# Autodesk Inventor assembly: tractionwheel_MIR
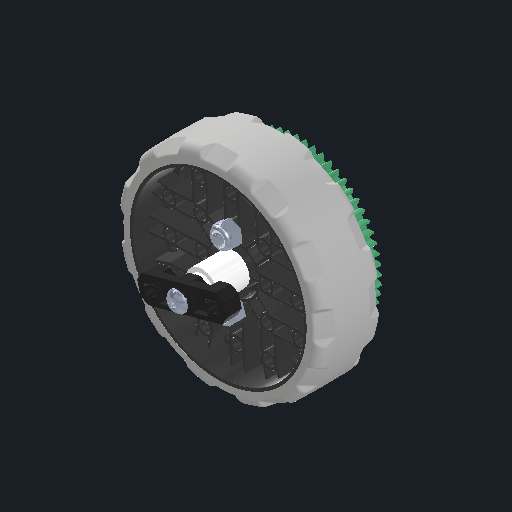
[picture p0: Inventor's stored thumbnail of the model, 512x512]
Saved by Autodesk Inventor 2024 (Build 280153000, 153)
## iProperties
Created: 2023-08-09
Part Number: tractionwheel_MIR
Document SubType Name: Assembly
Designer: macbook
Author: macbook
## Documents named in this file (16)
- \\Mac\Home\Desktop\code\1599V-VRC\Cad\Assembly\v3\tractionwheel_MIR.iam
- \\Mac\Home\Desktop\code\1599V-VRC\Cad\Motion\Shaft LS\Bearing Flat_MIR7.ipt
- \\Mac\Home\Desktop\code\1599V-VRC\Cad\Structure\Hardware\Screw Steel - Star\SScrew Star Threaded 1.250.ipt
- \\Mac\Home\Desktop\code\1599V-VRC\Cad\Structure\Hardware\Screw Steel - Star.ipt
- \\Mac\Home\Desktop\code\1599V-VRC\Cad\Structure\Hardware\Nut Nylock_MIR7.ipt
- \\Mac\Home\Desktop\code\1599V-VRC\Cad\Motion\Gears\LS 60T Gear_MIR5.ipt
- \\Mac\Home\Desktop\code\1599V-VRC\Cad\Structure\Hardware\Screw Steel - Star\SScrew Star Smooth 2.500.ipt
- \\Mac\Home\Desktop\code\1599V-VRC\Cad\Motion\Spacers\Spacer Nylon .500 OD\NSpacer White .500 OD x .500.ipt
- \\Mac\Home\Desktop\code\1599V-VRC\Cad\Motion\Spacers\Spacer Nylon .500 OD.ipt
- \\Mac\Home\Desktop\code\1599V-VRC\Cad\Motion\Spacers\Washer Steel\SWasher .375 OD x .015625.ipt
- \\Mac\Home\Desktop\code\1599V-VRC\Cad\Motion\Spacers\Washer Steel.ipt
- \\Mac\Home\Desktop\code\1599V-VRC\Cad\Motion\Spacers\Spacer Nylon .500 OD\NSpacer White .500 OD x .375.ipt
- \\Mac\Home\Desktop\code\1599V-VRC\Cad\Motion\Spacers\Washer Teflon\TWasher .375 OD x .03125.ipt
- \\Mac\Home\Desktop\code\1599V-VRC\Cad\Motion\Spacers\Washer Teflon.ipt
- \\Mac\Home\Desktop\code\1599V-VRC\Cad\Motion\Wheels\Traction Wheel\3.25 Traction AS, Circle_MIR2.iam
- \\Mac\Home\Desktop\code\1599V-VRC\Cad\Motion\Spacers\Washer Teflon\TWasher .375 OD x .06250.ipt
## Components (18 placed, 11 different names)
1. Bearing Flat_MIR7:1 — Insert:3, Insert:2, Insert:6
2. Bearing Flat_MIR7:2 — Insert:3, Insert:2, Insert:5, Insert:30
3. SScrew Star Threaded 1.250:1 — Insert:9
4. Nut Nylock_MIR7:1 — Insert:28
5. Nut Nylock_MIR7:2 — Insert:25
6. SScrew Star Threaded 1.250:2 — Insert:11
7. LS 60T Gear_MIR5:1 — Insert:29, Insert:10, Insert:12, Insert:13, Insert:27
8. SScrew Star Smooth 2.500:3 — Insert:5
9. Nut Nylock_MIR7:3 — Insert:6
10. NSpacer White .500 OD x .500:1 — Insert:22, Insert:26
11. SWasher .375 OD x .015625:1 — Insert:7
12. NSpacer White .500 OD x .375:2 — Insert:29, Insert:7, Insert:23
13. TWasher .375 OD x .03125:1 — Insert:10, Insert:9
14. TWasher .375 OD x .03125:2 — Insert:11, Insert:12
15. NSpacer White .500 OD x .375:3 — Insert:13, Insert:24
16. 3.25 Traction AS, Circle_MIR2:1 [sub-assembly] — Insert:28, Insert:25, Insert:24, Insert:23, Insert:22
17. TWasher .375 OD x .06250:3 — Insert:27
18. TWasher .375 OD x .06250:4 — Insert:30, Insert:26
## Relationships (19: Insert 19)
- Insert:3 (44.45 mm): Bearing Flat_MIR7:1 ↔ Bearing Flat_MIR7:2
- Insert:2 (44.45 mm): Bearing Flat_MIR7:1 ↔ Bearing Flat_MIR7:2
- Insert:5 (1.5875 mm): Bearing Flat_MIR7:2 ↔ SScrew Star Smooth 2.500:3
- Insert:6: Bearing Flat_MIR7:1 ↔ Nut Nylock_MIR7:3
- Insert:29: LS 60T Gear_MIR5:1 ↔ NSpacer White .500 OD x .375:2
- Insert:7: SWasher .375 OD x .015625:1 ↔ NSpacer White .500 OD x .375:2
- Insert:10: LS 60T Gear_MIR5:1 ↔ TWasher .375 OD x .03125:1
- Insert:9: SScrew Star Threaded 1.250:1 ↔ TWasher .375 OD x .03125:1
- Insert:11: SScrew Star Threaded 1.250:2 ↔ TWasher .375 OD x .03125:2
- Insert:12: LS 60T Gear_MIR5:1 ↔ TWasher .375 OD x .03125:2
- Insert:13: LS 60T Gear_MIR5:1 ↔ NSpacer White .500 OD x .375:3
- Insert:28: Nut Nylock_MIR7:1 ↔ 3.25 Traction AS, Circle_MIR2:1
- Insert:25: Nut Nylock_MIR7:2 ↔ 3.25 Traction AS, Circle_MIR2:1
- Insert:24: NSpacer White .500 OD x .375:3 ↔ 3.25 Traction AS, Circle_MIR2:1
- Insert:23: NSpacer White .500 OD x .375:2 ↔ 3.25 Traction AS, Circle_MIR2:1
- Insert:22: NSpacer White .500 OD x .500:1 ↔ 3.25 Traction AS, Circle_MIR2:1
- Insert:27: LS 60T Gear_MIR5:1 ↔ TWasher .375 OD x .06250:3
- Insert:30: Bearing Flat_MIR7:2 ↔ TWasher .375 OD x .06250:4
- Insert:26: NSpacer White .500 OD x .500:1 ↔ TWasher .375 OD x .06250:4
